# Autodesk Inventor assembly: main_pcb.brd
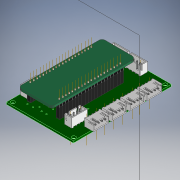
[picture p0: Inventor's stored thumbnail of the model, 180x180]
Saved by Autodesk Inventor 2022 (Build 260153000, 153)
## iProperties
Created: 2021-08-05
Part Number: main_pcb.brd
Document SubType Name: Assembly
Designer: Петров Иван
Mass: 18.6028 g
Surface Area: 275.031 cm^2
Volume: 13.5279 cm^3
Density: 1.37514 g/cm^3
Author: Петров Иван
## Documents named in this file (7)
- D:\IVAN\Ivan_desktop\Kvantorium\Projects\YouBotRobot\design\000.004 - Котроллер СНУ.iam
- D:\IVAN\Ivan_desktop\Kvantorium\Projects\YouBotRobot\design\standart_components\PBS-1.ipt
- D:\IVAN\Ivan_desktop\Kvantorium\Projects\YouBotRobot\design\standart_components\connectrs\JST - XH - Thru (R) - 4Pin - 2.54mm.ipt
- D:\IVAN\Ivan_desktop\Kvantorium\Projects\YouBotRobot\design\standart_components\connectrs\JST - XH - Thru (V) - 4Pin - 2.54mm.ipt
- D:\IVAN\Ivan_desktop\Kvantorium\Projects\YouBotRobot\design\000.004.001 - Плата печатная.ipt
- D:\IVAN\Ivan_desktop\Kvantorium\Projects\YouBotRobot\design\standart_components\CONN HEADER VERT 1POS 2.54MM.ipt
- D:\IVAN\Ivan_desktop\Kvantorium\Projects\YouBotRobot\design\standart_components\opencm904.ipt
## Components (90 placed, 6 different names)
1. 000.004.001 - Плата печатная — Совмещение:15, Совмещение:16, Совмещение:17, Совмещение:18, Совмещение:19, Совмещение:20, Совмещение:26, Совмещение:27, Совмещение:28, Совмещение:29, Совмещение:30, Совмещение:31
2. JST - XH - Thru (R) - 4Pin - 2.54mm:1
3. JST - XH - Thru (R) - 4Pin - 2.54mm:2
4. JST - XH - Thru (V) - 4Pin - 2.54mm:1
5. JST - XH - Thru (V) - 4Pin - 2.54mm:2
6. JST - XH - Thru (R) - 4Pin - 2.54mm:3 — Совмещение:18, Совмещение:19, Совмещение:20
7. JST - XH - Thru (R) - 4Pin - 2.54mm:4 — Совмещение:15, Совмещение:16, Совмещение:17
8. untitled.brdКонтур:1 — Совмещение:23, Совмещение:24, Совмещение:25
9. JST - XH - Thru (V) - 4Pin - 2.54mm:3 — Совмещение:26, Совмещение:27, Совмещение:28
10. JST - XH - Thru (V) - 4Pin - 2.54mm:4 — Совмещение:29, Совмещение:30, Совмещение:31
11. PBS-1:2 — Совмещение:21, Совмещение:22, Заподлицо:1
12. PBS-1:3
13. PBS-1:4
14. PBS-1:5
15. PBS-1:6
16. PBS-1:7
17. PBS-1:8
18. PBS-1:9
19. PBS-1:10
20. PBS-1:11
21. PBS-1:12
22. PBS-1:13
23. PBS-1:14
24. PBS-1:15
25. PBS-1:16
26. PBS-1:17
27. PBS-1:18
28. PBS-1:19
29. PBS-1:20
30. PBS-1:21
31. PBS-1:22
32. PBS-1:23
33. PBS-1:24
34. PBS-1:25
35. PBS-1:26
36. PBS-1:27
37. PBS-1:28
38. PBS-1:29
39. PBS-1:30
40. PBS-1:31
41. PBS-1:32
42. PBS-1:33
43. PBS-1:34
44. PBS-1:35
45. PBS-1:36
46. PBS-1:37
47. PBS-1:38
48. PBS-1:39
49. PBS-1:40
50. PBS-1:41
51. CONN HEADER VERT 1POS 2.54MM:1 — Совмещение:21, Совмещение:22, Заподлицо:1, Совмещение:23, Совмещение:24
52. CONN HEADER VERT 1POS 2.54MM:2
53. CONN HEADER VERT 1POS 2.54MM:3
54. CONN HEADER VERT 1POS 2.54MM:4
55. CONN HEADER VERT 1POS 2.54MM:5
56. CONN HEADER VERT 1POS 2.54MM:6
57. CONN HEADER VERT 1POS 2.54MM:7
58. CONN HEADER VERT 1POS 2.54MM:8
59. CONN HEADER VERT 1POS 2.54MM:9
60. CONN HEADER VERT 1POS 2.54MM:10
61. CONN HEADER VERT 1POS 2.54MM:11
62. CONN HEADER VERT 1POS 2.54MM:12
63. CONN HEADER VERT 1POS 2.54MM:13
64. CONN HEADER VERT 1POS 2.54MM:14
65. CONN HEADER VERT 1POS 2.54MM:15
66. CONN HEADER VERT 1POS 2.54MM:16
67. CONN HEADER VERT 1POS 2.54MM:17
68. CONN HEADER VERT 1POS 2.54MM:18
69. CONN HEADER VERT 1POS 2.54MM:19
70. CONN HEADER VERT 1POS 2.54MM:20
71. CONN HEADER VERT 1POS 2.54MM:21
72. CONN HEADER VERT 1POS 2.54MM:22
73. CONN HEADER VERT 1POS 2.54MM:23
74. CONN HEADER VERT 1POS 2.54MM:24
75. CONN HEADER VERT 1POS 2.54MM:25
76. CONN HEADER VERT 1POS 2.54MM:26
77. CONN HEADER VERT 1POS 2.54MM:27
78. CONN HEADER VERT 1POS 2.54MM:28
79. CONN HEADER VERT 1POS 2.54MM:29
80. CONN HEADER VERT 1POS 2.54MM:30
81. CONN HEADER VERT 1POS 2.54MM:31
82. CONN HEADER VERT 1POS 2.54MM:32
83. CONN HEADER VERT 1POS 2.54MM:33
84. CONN HEADER VERT 1POS 2.54MM:34
85. CONN HEADER VERT 1POS 2.54MM:35
86. CONN HEADER VERT 1POS 2.54MM:36
87. CONN HEADER VERT 1POS 2.54MM:37
88. CONN HEADER VERT 1POS 2.54MM:38
89. CONN HEADER VERT 1POS 2.54MM:39
90. CONN HEADER VERT 1POS 2.54MM:40 — Совмещение:25
## Component patterns: (40 elements, first: PBS-1:2), (40 elements, first: CONN HEADER VERT 1POS 2.54MM:1)
## Relationships (33: Mate 31, Angle 1, Flush 1)
- [Mate]: 000.004.001 - Плата печатная ↔ PBS-1:2
- [Angle] (90 deg): 000.004.001 - Плата печатная ↔ PBS-1:2
- [Mate]: 000.004.001 - Плата печатная ↔ PBS-1:2
- [Mate]: 000.004.001 - Плата печатная ↔ JST - XH - Thru (R) - 4Pin - 2.54mm:1
- [Mate]: 000.004.001 - Плата печатная ↔ JST - XH - Thru (R) - 4Pin - 2.54mm:1
- [Mate]: 000.004.001 - Плата печатная ↔ JST - XH - Thru (R) - 4Pin - 2.54mm:1
- [Mate]: 000.004.001 - Плата печатная ↔ JST - XH - Thru (R) - 4Pin - 2.54mm:2
- [Mate]: 000.004.001 - Плата печатная ↔ JST - XH - Thru (R) - 4Pin - 2.54mm:2
- [Mate]: 000.004.001 - Плата печатная ↔ JST - XH - Thru (R) - 4Pin - 2.54mm:2
- [Mate]: 000.004.001 - Плата печатная ↔ JST - XH - Thru (V) - 4Pin - 2.54mm:1
- [Mate]: 000.004.001 - Плата печатная ↔ JST - XH - Thru (V) - 4Pin - 2.54mm:1
- [Mate]: 000.004.001 - Плата печатная ↔ JST - XH - Thru (V) - 4Pin - 2.54mm:1
- [Mate]: 000.004.001 - Плата печатная ↔ JST - XH - Thru (V) - 4Pin - 2.54mm:2
- [Mate]: 000.004.001 - Плата печатная ↔ JST - XH - Thru (V) - 4Pin - 2.54mm:2
- [Mate]: 000.004.001 - Плата печатная ↔ JST - XH - Thru (V) - 4Pin - 2.54mm:2
- Совмещение:15 [Mate]: 000.004.001 - Плата печатная ↔ JST - XH - Thru (R) - 4Pin - 2.54mm:4
- Совмещение:16 [Mate]: 000.004.001 - Плата печатная ↔ JST - XH - Thru (R) - 4Pin - 2.54mm:4
- Совмещение:17 [Mate]: 000.004.001 - Плата печатная ↔ JST - XH - Thru (R) - 4Pin - 2.54mm:4
- Совмещение:18 [Mate]: 000.004.001 - Плата печатная ↔ JST - XH - Thru (R) - 4Pin - 2.54mm:3
- Совмещение:19 [Mate]: 000.004.001 - Плата печатная ↔ JST - XH - Thru (R) - 4Pin - 2.54mm:3
- Совмещение:20 [Mate]: 000.004.001 - Плата печатная ↔ JST - XH - Thru (R) - 4Pin - 2.54mm:3
- Совмещение:21 [Mate]: PBS-1:2 ↔ CONN HEADER VERT 1POS 2.54MM:1
- Совмещение:22 [Mate]: PBS-1:2 ↔ CONN HEADER VERT 1POS 2.54MM:1
- Заподлицо:1 [Flush]: PBS-1:2 ↔ CONN HEADER VERT 1POS 2.54MM:1
- Совмещение:23 [Mate]: untitled.brdКонтур:1 ↔ CONN HEADER VERT 1POS 2.54MM:1
- Совмещение:24 [Mate]: untitled.brdКонтур:1 ↔ CONN HEADER VERT 1POS 2.54MM:1
- Совмещение:25 [Mate]: untitled.brdКонтур:1 ↔ CONN HEADER VERT 1POS 2.54MM:40
- Совмещение:26 [Mate]: 000.004.001 - Плата печатная ↔ JST - XH - Thru (V) - 4Pin - 2.54mm:3
- Совмещение:27 [Mate]: 000.004.001 - Плата печатная ↔ JST - XH - Thru (V) - 4Pin - 2.54mm:3
- Совмещение:28 [Mate]: 000.004.001 - Плата печатная ↔ JST - XH - Thru (V) - 4Pin - 2.54mm:3
- Совмещение:29 [Mate]: 000.004.001 - Плата печатная ↔ JST - XH - Thru (V) - 4Pin - 2.54mm:4
- Совмещение:30 [Mate]: 000.004.001 - Плата печатная ↔ JST - XH - Thru (V) - 4Pin - 2.54mm:4
- Совмещение:31 [Mate]: 000.004.001 - Плата печатная ↔ JST - XH - Thru (V) - 4Pin - 2.54mm:4
